# Autodesk Inventor assembly: Main_Assembly
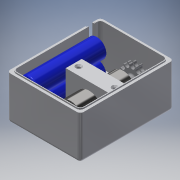
[picture p0: Inventor's stored thumbnail of the model, 180x180]
Saved by Autodesk Inventor 2017 (Build 210142000, 142)
## iProperties
Created: 2018-10-14
Part Number: Main_Assembly
Document SubType Name: Assembly
Designer: Mitch
Author: Mitch
## Documents named in this file (6)
- E:\Youtube Channel\Pojects\Chain Blinds\Mechanical\Main_Assembly.iam
- E:\Youtube Channel\Pojects\Chain Blinds\Mechanical\Case_Bottom.ipt
- E:\Youtube Channel\Pojects\Chain Blinds\Mechanical\Motor.ipt
- E:\Youtube Channel\Pojects\Chain Blinds\Mechanical\battery pack.iam
- E:\Youtube Channel\Pojects\Chain Blinds\Mechanical\chain_gear.ipt
- E:\Youtube Channel\Pojects\Chain Blinds\Mechanical\Motor_Mount_Top.ipt
## Components (5 placed, 5 different names)
1. Case_Bottom:1 — Mate:3, Mate:4, Mate:5, Tangent:1, Tangent:2, Tangent:3, Mate:6, Mate:7
2. Motor:1 — Mate:1, Mate:2, Mate:3, Mate:4
3. battery pack:1 [sub-assembly] — Mate:5, Tangent:1, Tangent:2, Tangent:3
4. chain_gear:1 — Mate:1, Mate:2
5. Motor_Mount_Top:1 — Mate:6, Mate:7
## Relationships (10: Mate 7, Tangent 3)
- Mate:1: Motor:1 ↔ chain_gear:1
- Mate:2: Motor:1 ↔ chain_gear:1
- Mate:3 (3.81 mm): Case_Bottom:1 ↔ Motor:1
- Mate:4: Case_Bottom:1 ↔ Motor:1
- Mate:5 (5.08 mm): Case_Bottom:1 ↔ battery pack:1
- Tangent:1: Case_Bottom:1 ↔ battery pack:1
- Tangent:2: Case_Bottom:1 ↔ battery pack:1
- Tangent:3: Case_Bottom:1 ↔ battery pack:1
- Mate:6: Case_Bottom:1 ↔ Motor_Mount_Top:1
- Mate:7: Case_Bottom:1 ↔ Motor_Mount_Top:1
